# Autodesk Inventor assembly: Rebuild Electrical Board 1
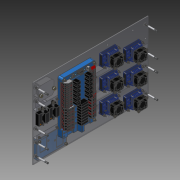
[picture p0: Inventor's stored thumbnail of the model, 180x180]
Saved by Autodesk Inventor 2014 SP1 (Build 180222100, 222)
## iProperties
Created: 2013-01-27
Part Number: Rebuild Electrical Board 1
Document SubType Name: Assembly
Designer: Moses
Mass: 4890.59 g
Surface Area: 13907.1 cm^2
Volume: 1924.91 cm^3
Density: 2.54069 g/cm^3
Author: Moses
## Documents named in this file (25)
- C:\Users\Moses\Documents\Inventor\Sally Rebuild\Rebuild Sally\Rebuild Electrical Board 1.iam
- C:\Users\Moses\Documents\Inventor\Sally Rebuild\Rebuild Sally\CS_PowerBoard_A003206.ipt
- C:\Users\Moses\Documents\Inventor\Sally Rebuild\Rebuild Sally\CS_Converter_CLL25-24S05.ipt
- C:\Users\Moses\Documents\Inventor\Sally Rebuild\Rebuild Sally\93330A493.ipt
- C:\Users\Moses\Documents\Inventor\Sally Rebuild\Rebuild Sally\CS_Relay_SPIKE-RELAY-H.ipt
- C:\Users\Moses\Documents\Inventor\Sally Rebuild\Rebuild Sally\Talon with Fan.iam
- C:\Users\Moses\Documents\Inventor\Sally Rebuild\Rebuild Sally\CS_SideCar_A003333.ipt
- C:\Users\Moses\Documents\Inventor\Sally Rebuild\Rebuild Sally\Rebuild Mounting Board 1.ipt
- C:\Users\Moses\Documents\Inventor\Sally Rebuild\Rebuild Sally\Electrical Board 1 Bracing L Channel.ipt
- C:\Users\Moses\Documents\Inventor\Sally Rebuild\Rebuild Sally\Electrical Board 1 Bracing L Channel Part 2.ipt
- C:\Users\Moses\Documents\Inventor\Sally Rebuild\Rebuild Sally\Pneumatics\Pneumatics_Clippard_AVT-32-32.iam
- C:\Users\Moses\Documents\Inventor\Sally Rebuild\Rebuild Sally\Pneumatics\Pneumatics_SMC_KQ2H07-35S.ipt
- C:\Users\Moses\Documents\Inventor\Sally Rebuild\Rebuild Sally\Standard #10 Washer.ipt
- C:\Users\Moses\Documents\Inventor\Sally Rebuild\Rebuild Sally\10-32 316 Stainless Steel Pan Head Philips Machine Screw\0.500\91735A829.ipt
- C:\Users\Moses\Documents\Inventor\Sally Rebuild\Rebuild Sally\90715A007.ipt
- C:\Users\Moses\Documents\Inventor\Sally Rebuild\Rebuild Sally\6-32 18-8 Stainless Steel Pan Head Philips Machine Screw\0.6250\91772A150.ipt
- C:\Users\Moses\Documents\Inventor\Sally Rebuild\Rebuild Sally\6-32 18-8 Stainless Steel Pan Head Philips Machine Screw\1.0000\91772A153.ipt
- C:\Users\Moses\Documents\Inventor\Sally Rebuild\Rebuild Sally\10-32 316 Stainless Steel Pan Head Philips Machine Screw\0.625\91735A830.ipt
- C:\Users\Moses\Documents\Inventor\Sally Rebuild\Rebuild Sally\6-32 18-8 Stainless Steel Pan Head Philips Machine Screw\1.2500\91772A155.ipt
- C:\Users\Moses\Documents\Inventor\Sally Rebuild\Rebuild Sally\91831A411.ipt
- C:\Users\Moses\Documents\Inventor\Sally Rebuild\Rebuild Sally\Standard #4 Washer.ipt
- C:\Users\Moses\Documents\Inventor\Sally Rebuild\Rebuild Sally\4-40 18-8 Stainless Steel Pan Head Phillips Machine Screw\0.5000\91772A110.ipt
- C:\Users\Moses\Documents\Inventor\Sally Rebuild\Rebuild Sally\4-40 18-8 Stainless Steel Pan Head Phillips Machine Screw\1.1250\91772A118.ipt
- C:\Users\Moses\Documents\Inventor\Sally Rebuild\Rebuild Sally\4-40 18-8 Stainless Steel Pan Head Phillips Machine Screw\18-8 Stainless Steel Machine Screw Hex Nut\91841A005.ipt
- C:\Users\Moses\Documents\Inventor\Sally Rebuild\Rebuild Sally\Standard #6 Washer.ipt
## Components (153 placed, 24 different names)
1. Rebuild Mounting Board 1:1 — Mate:1, Mate:2, Mate:3, Mate:4, Mate:5, Mate:6, Mate:7, Mate:8, Mate:9, Mate:10, Mate:11, Mate:12, Mate:13, Mate:14, Mate:15, Mate:16, Mate:17, Mate:18, Mate:19, Mate:20, Mate:21, Mate:22, Mate:23, Mate:24, Mate:25, Mate:26, Insert:2, Insert:4, Insert:5, Insert:7, Insert:8, Mate:27, Mate:28, Mate:29, Mate:30, Mate:31, Mate:32, Mate:33, Mate:34, Mate:35, Insert:9, Insert:10, Insert:11, Insert:13, Mate:36, Mate:37, Flush:1, Flush:2, Tangent:1, Tangent:2, Flush:5, Flush:6, Mate:38, Mate:39, Insert:18, Insert:19, Insert:20, Insert:21, Insert:22, Insert:23, Insert:24, Insert:25, Insert:26, Angle:3, Angle:4, Insert:90, Insert:91
2. Talon with Fan:1 [sub-assembly] — Mate:1, Mate:6, Mate:7
3. Talon with Fan:2 [sub-assembly] — Mate:2, Mate:8, Mate:9
4. Talon with Fan:3 [sub-assembly] — Mate:3, Mate:10, Mate:11
5. Talon with Fan:4 [sub-assembly] — Mate:4, Mate:12, Mate:13
6. Talon with Fan:5 [sub-assembly] — Mate:14, Mate:15, Mate:16
7. Talon with Fan:6 [sub-assembly] — Mate:5, Mate:17, Mate:18
8. CS_PowerBoard_A003206:1 — Mate:19, Mate:20, Mate:21, Mate:22, Mate:23
9. CS_Converter_CLL25-24S05:1 — Mate:24, Mate:25, Mate:26, Insert:137, Insert:138
10. CS_Relay_SPIKE-RELAY-H:1 — Mate:28, Mate:29, Mate:30
11. CS_Relay_SPIKE-RELAY-H:2 — Mate:27, Mate:31, Mate:32
12. CS_SideCar_A003333:1 — Mate:33, Mate:34, Mate:35
13. Electrical Board 1 Bracing L Channel:1 — Mate:36, Flush:2, Angle:1, Tangent:3, Mate:38, Insert:167
14. Electrical Board 1 Bracing L Channel Part 2:1 — Mate:37, Flush:1, Angle:2, Tangent:4, Mate:39
15. Pneumatics_Clippard_AVT-32-32:1 [sub-assembly] — Tangent:2, Angle:1, Tangent:3, Flush:6, Insert:15, Insert:17, Angle:3
16. Pneumatics_Clippard_AVT-32-32:2 [sub-assembly] — Tangent:1, Angle:2, Tangent:4, Flush:5, Insert:14, Insert:16, Angle:4
17. Pneumatics_SMC_KQ2H07-35S:1 — Insert:14
18. Pneumatics_SMC_KQ2H07-35S:2 — Insert:15
19. Pneumatics_SMC_KQ2H07-35S:3 — Insert:16
20. Pneumatics_SMC_KQ2H07-35S:4 — Insert:17
21. Standard #4 Washer:50 — Insert:133, Insert:167
22. 91841A005:1 — Insert:145
23. 91841A005:2 — Insert:146
24. 91841A005:3 — Insert:147
25. 91841A005:5 — Insert:149
26. 91841A005:4 — Insert:148
27. 91841A005:6 — Insert:150
28. 91841A005:7 — Insert:151
29. 91841A005:8 — Insert:152
30. 91841A005:10 — Insert:153
31. 91841A005:9 — Insert:154
32. 91772A118:2 — Insert:156
33. 91772A118:1 — Insert:155
34. 91772A118:4 — Insert:158
35. 91772A118:3 — Insert:157
36. 91772A118:6 — Insert:160
37. 91772A118:5 — Insert:159
38. 91772A118:7 — Insert:161
39. 91772A118:9 — Insert:163
40. 91772A118:8 — Insert:162
41. 91772A118:10 — Insert:164
42. 91772A118:12 — Insert:166
43. 91772A118:11 — Insert:165
44. 93330A493:2 — Insert:2
45. 93330A493:4 — Insert:4
46. 93330A493:5 — Insert:5
47. 93330A493:7 — Insert:7
48. 93330A493:8 — Insert:8
49. 93330A493:9 — Insert:10
50. 93330A493:11 — Insert:11
51. 93330A493:10 — Insert:9
52. 93330A493:13 — Insert:13
53. 91772A110:1
54. 91772A110:3
55. 91772A110:2
56. 91772A110:4
57. 91772A110:5
58. 91772A110:6
59. 91772A110:7 — Insert:133
60. 91772A110:10
61. 91772A110:8
62. 91772A110:9
63. 91735A830:1 — Insert:137
64. 91735A830:2 — Insert:138
65. 91772A155:1
66. 91772A155:2
67. Standard #4 Washer:49
68. 91772A155:3
69. 91831A411:1 — Insert:143
70. 91831A411:2 — Insert:144
71. 90715A007:5
72. 90715A007:6
73. 90715A007:7
74. 90715A007:8
75. 91772A150:1
76. 91772A150:2
77. 91772A150:3
78. 91772A150:4
79. 90715A007:9
80. 90715A007:11
81. Standard #6 Washer:1
82. Standard #6 Washer:2
83. 91772A153:1
84. 91772A153:2
85. Standard #4 Washer:39 — Insert:151
86. Standard #4 Washer:40 — Insert:152
87. Standard #4 Washer:41 — Insert:154
88. Standard #4 Washer:42 — Insert:153
89. Standard #4 Washer:43 — Insert:145
90. Standard #4 Washer:44 — Insert:150
91. Standard #4 Washer:45 — Insert:146
92. Standard #4 Washer:46 — Insert:149
93. Standard #4 Washer:47 — Insert:148
94. Standard #4 Washer:48 — Insert:147
95. 90715A007:2
96. 90715A007:1
97. 90715A007:4
98. Standard #4 Washer:25 — Insert:157
99. Standard #4 Washer:26 — Insert:158
100. Standard #4 Washer:27 — Insert:155
101. Standard #4 Washer:28 — Insert:156
102. Standard #4 Washer:29 — Insert:161
103. Standard #4 Washer:30 — Insert:162
104. Standard #4 Washer:31 — Insert:160
105. Standard #4 Washer:32 — Insert:159
106. Standard #4 Washer:33 — Insert:164
107. Standard #4 Washer:34 — Insert:163
108. Standard #4 Washer:35 — Insert:166
109. Standard #4 Washer:36 — Insert:165
110. Standard #10 Washer:10 — Insert:91, Insert:143
111. Standard #10 Washer:11 — Insert:90, Insert:144
112. Standard #4 Washer:1
113. Standard #4 Washer:2
114. Standard #4 Washer:3
115. Standard #4 Washer:4
116. Standard #4 Washer:5
117. Standard #4 Washer:6
118. Standard #6 Washer:15
119. Standard #4 Washer:8
120. Standard #6 Washer:12
121. Standard #4 Washer:11
122. Standard #4 Washer:10
123. Standard #6 Washer:8
124. Standard #6 Washer:9
125. Standard #6 Washer:10
126. Standard #6 Washer:11
127. Standard #6 Washer:13
128. Standard #6 Washer:14
129. Standard #6 Washer:7
130. Standard #6 Washer:6
131. Standard #6 Washer:5
132. Standard #6 Washer:4
133. Standard #6 Washer:3
134. Standard #4 Washer:23
135. Standard #4 Washer:24
136. Standard #10 Washer:1 — Insert:18, Insert:27
137. Standard #10 Washer:2 — Insert:19, Insert:28
138. Standard #10 Washer:3 — Insert:20, Insert:29
139. Standard #10 Washer:5 — Insert:22, Insert:31
140. Standard #10 Washer:4 — Insert:21, Insert:30
141. Standard #10 Washer:6 — Insert:23, Insert:32
142. Standard #10 Washer:7 — Insert:24, Insert:33
143. Standard #10 Washer:8 — Insert:25, Insert:34
144. Standard #10 Washer:9 — Insert:26, Insert:35
145. 91735A829:1 — Insert:27
146. 91735A829:2 — Insert:28
147. 91735A829:3 — Insert:29
148. 91735A829:4 — Insert:30
149. 91735A829:5 — Insert:31
150. 91735A829:7 — Insert:33
151. 91735A829:6 — Insert:32
152. 91735A829:8 — Insert:34
153. 91735A829:9 — Insert:35
## Relationships (188: Insert 137, Mate 39, Flush 4, Tangent 4, Angle 4)
- Mate:1: Rebuild Mounting Board 1:1 ↔ Talon with Fan:1
- Mate:2: Rebuild Mounting Board 1:1 ↔ Talon with Fan:2
- Mate:3: Rebuild Mounting Board 1:1 ↔ Talon with Fan:3
- Mate:4: Rebuild Mounting Board 1:1 ↔ Talon with Fan:4
- Mate:5: Rebuild Mounting Board 1:1 ↔ Talon with Fan:6
- Mate:6: Rebuild Mounting Board 1:1 ↔ Talon with Fan:1
- Mate:7: Rebuild Mounting Board 1:1 ↔ Talon with Fan:1
- Mate:8: Rebuild Mounting Board 1:1 ↔ Talon with Fan:2
- Mate:9: Rebuild Mounting Board 1:1 ↔ Talon with Fan:2
- Mate:10: Rebuild Mounting Board 1:1 ↔ Talon with Fan:3
- Mate:11: Rebuild Mounting Board 1:1 ↔ Talon with Fan:3
- Mate:12: Rebuild Mounting Board 1:1 ↔ Talon with Fan:4
- Mate:13: Rebuild Mounting Board 1:1 ↔ Talon with Fan:4
- Mate:14: Rebuild Mounting Board 1:1 ↔ Talon with Fan:5
- Mate:15: Rebuild Mounting Board 1:1 ↔ Talon with Fan:5
- Mate:16: Rebuild Mounting Board 1:1 ↔ Talon with Fan:5
- Mate:17: Rebuild Mounting Board 1:1 ↔ Talon with Fan:6
- Mate:18: Rebuild Mounting Board 1:1 ↔ Talon with Fan:6
- Mate:19: Rebuild Mounting Board 1:1 ↔ CS_PowerBoard_A003206:1
- Mate:20: Rebuild Mounting Board 1:1 ↔ CS_PowerBoard_A003206:1
- Mate:21: Rebuild Mounting Board 1:1 ↔ CS_PowerBoard_A003206:1
- Mate:22: Rebuild Mounting Board 1:1 ↔ CS_PowerBoard_A003206:1
- Mate:23: Rebuild Mounting Board 1:1 ↔ CS_PowerBoard_A003206:1
- Mate:24: Rebuild Mounting Board 1:1 ↔ CS_Converter_CLL25-24S05:1
- Mate:25: Rebuild Mounting Board 1:1 ↔ CS_Converter_CLL25-24S05:1
- Mate:26: Rebuild Mounting Board 1:1 ↔ CS_Converter_CLL25-24S05:1
- Insert:2: Rebuild Mounting Board 1:1 ↔ 93330A493:2
- Insert:4: Rebuild Mounting Board 1:1 ↔ 93330A493:4
- Insert:5: Rebuild Mounting Board 1:1 ↔ 93330A493:5
- Insert:7: Rebuild Mounting Board 1:1 ↔ 93330A493:7
- Insert:8: Rebuild Mounting Board 1:1 ↔ 93330A493:8
- Mate:27: Rebuild Mounting Board 1:1 ↔ CS_Relay_SPIKE-RELAY-H:2
- Mate:28: Rebuild Mounting Board 1:1 ↔ CS_Relay_SPIKE-RELAY-H:1
- Mate:29: Rebuild Mounting Board 1:1 ↔ CS_Relay_SPIKE-RELAY-H:1
- Mate:30: Rebuild Mounting Board 1:1 ↔ CS_Relay_SPIKE-RELAY-H:1
- Mate:31: Rebuild Mounting Board 1:1 ↔ CS_Relay_SPIKE-RELAY-H:2
- Mate:32: Rebuild Mounting Board 1:1 ↔ CS_Relay_SPIKE-RELAY-H:2
- Mate:33: Rebuild Mounting Board 1:1 ↔ CS_SideCar_A003333:1
- Mate:34: Rebuild Mounting Board 1:1 ↔ CS_SideCar_A003333:1
- Mate:35: Rebuild Mounting Board 1:1 ↔ CS_SideCar_A003333:1
- Insert:9: Rebuild Mounting Board 1:1 ↔ 93330A493:10
- Insert:10: Rebuild Mounting Board 1:1 ↔ 93330A493:9
- Insert:11: Rebuild Mounting Board 1:1 ↔ 93330A493:11
- Insert:13: Rebuild Mounting Board 1:1 ↔ 93330A493:13
- Mate:36: Rebuild Mounting Board 1:1 ↔ Electrical Board 1 Bracing L Channel:1
- Mate:37: Rebuild Mounting Board 1:1 ↔ Electrical Board 1 Bracing L Channel Part 2:1
- Flush:1: Rebuild Mounting Board 1:1 ↔ Electrical Board 1 Bracing L Channel Part 2:1
- Flush:2: Rebuild Mounting Board 1:1 ↔ Electrical Board 1 Bracing L Channel:1
- Tangent:1 (3.81 mm): Rebuild Mounting Board 1:1 ↔ Pneumatics_Clippard_AVT-32-32:2
- Tangent:2: Rebuild Mounting Board 1:1 ↔ Pneumatics_Clippard_AVT-32-32:1
- Angle:1 (0 deg): Electrical Board 1 Bracing L Channel:1 ↔ Pneumatics_Clippard_AVT-32-32:1
- Angle:2 (0 deg): Electrical Board 1 Bracing L Channel Part 2:1 ↔ Pneumatics_Clippard_AVT-32-32:2
- Tangent:3: Electrical Board 1 Bracing L Channel:1 ↔ Pneumatics_Clippard_AVT-32-32:1
- Tangent:4: Electrical Board 1 Bracing L Channel Part 2:1 ↔ Pneumatics_Clippard_AVT-32-32:2
- Flush:5 (25.4 mm): Rebuild Mounting Board 1:1 ↔ Pneumatics_Clippard_AVT-32-32:2
- Flush:6 (127 mm): Rebuild Mounting Board 1:1 ↔ Pneumatics_Clippard_AVT-32-32:1
- Insert:14 (1.27 mm): Pneumatics_Clippard_AVT-32-32:2 ↔ Pneumatics_SMC_KQ2H07-35S:1
- Insert:15 (1.27 mm): Pneumatics_Clippard_AVT-32-32:1 ↔ Pneumatics_SMC_KQ2H07-35S:2
- Insert:16 (1.27 mm): Pneumatics_Clippard_AVT-32-32:2 ↔ Pneumatics_SMC_KQ2H07-35S:3
- Insert:17 (1.27 mm): Pneumatics_Clippard_AVT-32-32:1 ↔ Pneumatics_SMC_KQ2H07-35S:4
- Mate:38: Rebuild Mounting Board 1:1 ↔ Electrical Board 1 Bracing L Channel:1
- Mate:39: Rebuild Mounting Board 1:1 ↔ Electrical Board 1 Bracing L Channel Part 2:1
- Insert:18: Rebuild Mounting Board 1:1 ↔ Standard #10 Washer:1
- Insert:19: Rebuild Mounting Board 1:1 ↔ Standard #10 Washer:2
- Insert:20: Rebuild Mounting Board 1:1 ↔ Standard #10 Washer:3
- Insert:21: Rebuild Mounting Board 1:1 ↔ Standard #10 Washer:4
- Insert:22: Rebuild Mounting Board 1:1 ↔ Standard #10 Washer:5
- Insert:23: Rebuild Mounting Board 1:1 ↔ Standard #10 Washer:6
- Insert:24: Rebuild Mounting Board 1:1 ↔ Standard #10 Washer:7
- Insert:25: Rebuild Mounting Board 1:1 ↔ Standard #10 Washer:8
- Insert:26: Rebuild Mounting Board 1:1 ↔ Standard #10 Washer:9
- Insert:27: Standard #10 Washer:1 ↔ 91735A829:1
- Insert:28: Standard #10 Washer:2 ↔ 91735A829:2
- Insert:29: Standard #10 Washer:3 ↔ 91735A829:3
- Insert:30: Standard #10 Washer:4 ↔ 91735A829:4
- Insert:31: Standard #10 Washer:5 ↔ 91735A829:5
- Insert:32: Standard #10 Washer:6 ↔ 91735A829:6
- Insert:33: Standard #10 Washer:7 ↔ 91735A829:7
- Insert:34: Standard #10 Washer:8 ↔ 91735A829:8
- Insert:35: Standard #10 Washer:9 ↔ 91735A829:9
- Angle:3 (0 deg): Rebuild Mounting Board 1:1 ↔ Pneumatics_Clippard_AVT-32-32:1
- Angle:4 (0 deg): Rebuild Mounting Board 1:1 ↔ Pneumatics_Clippard_AVT-32-32:2
- [Insert]: Electrical Board 1 Bracing L Channel:1 ↔ Standard #4 Washer:1
- [Insert]: Electrical Board 1 Bracing L Channel:1 ↔ Standard #4 Washer:2
- [Insert]: Electrical Board 1 Bracing L Channel:1 ↔ Standard #4 Washer:3
- [Insert]: Electrical Board 1 Bracing L Channel Part 2:1 ↔ Standard #4 Washer:4
- [Insert]: Electrical Board 1 Bracing L Channel Part 2:1 ↔ Standard #4 Washer:5
- [Insert]: Electrical Board 1 Bracing L Channel Part 2:1 ↔ Standard #4 Washer:6
- [Insert]: Electrical Board 1 Bracing L Channel:1 ↔ Standard #6 Washer:15
- [Insert]: Electrical Board 1 Bracing L Channel:1 ↔ Standard #4 Washer:8
- [Insert]: Electrical Board 1 Bracing L Channel:1 ↔ Standard #6 Washer:12
- [Insert]: Electrical Board 1 Bracing L Channel Part 2:1 ↔ Standard #4 Washer:10
- [Insert]: Electrical Board 1 Bracing L Channel Part 2:1 ↔ Standard #4 Washer:11
- [Insert]: CS_Relay_SPIKE-RELAY-H:1 ↔ Standard #6 Washer:8
- [Insert]: CS_Relay_SPIKE-RELAY-H:2 ↔ Standard #6 Washer:9
- [Insert]: CS_Relay_SPIKE-RELAY-H:1 ↔ Standard #6 Washer:11
- [Insert]: CS_Relay_SPIKE-RELAY-H:2 ↔ Standard #6 Washer:10
- [Insert]: Rebuild Mounting Board 1:1 ↔ Standard #6 Washer:13
- [Insert]: Rebuild Mounting Board 1:1 ↔ Standard #6 Washer:14
- [Insert]: Rebuild Mounting Board 1:1 ↔ Standard #6 Washer:7
- [Insert]: Rebuild Mounting Board 1:1 ↔ Standard #6 Washer:6
- [Insert]: CS_PowerBoard_A003206:1 ↔ Standard #6 Washer:5
- [Insert]: CS_PowerBoard_A003206:1 ↔ Standard #6 Washer:4
- [Insert]: CS_PowerBoard_A003206:1 ↔ Standard #6 Washer:3
- [Insert]: Rebuild Mounting Board 1:1 ↔ Standard #4 Washer:23
- [Insert]: Rebuild Mounting Board 1:1 ↔ Standard #4 Washer:24
- [Insert]: 90715A007:1 ↔ Standard #6 Washer:3
- [Insert]: 90715A007:2 ↔ Standard #6 Washer:4
- [Insert]: 90715A007:4 ↔ Standard #6 Washer:5
- [Insert]: Rebuild Mounting Board 1:1 ↔ Standard #4 Washer:25
- [Insert]: Electrical Board 1 Bracing L Channel:1 ↔ Standard #4 Washer:26
- [Insert]: Rebuild Mounting Board 1:1 ↔ Standard #4 Washer:27
- [Insert]: Rebuild Mounting Board 1:1 ↔ Standard #4 Washer:28
- [Insert]: Rebuild Mounting Board 1:1 ↔ Standard #4 Washer:29
- [Insert]: Rebuild Mounting Board 1:1 ↔ Standard #4 Washer:30
- [Insert]: Rebuild Mounting Board 1:1 ↔ Standard #4 Washer:31
- [Insert]: Rebuild Mounting Board 1:1 ↔ Standard #4 Washer:32
- [Insert]: Rebuild Mounting Board 1:1 ↔ Standard #4 Washer:33
- [Insert]: Rebuild Mounting Board 1:1 ↔ Standard #4 Washer:34
- [Insert]: Rebuild Mounting Board 1:1 ↔ Standard #4 Washer:35
- [Insert]: Electrical Board 1 Bracing L Channel Part 2:1 ↔ Standard #4 Washer:36
- Insert:90: Rebuild Mounting Board 1:1 ↔ Standard #10 Washer:11
- Insert:91: Rebuild Mounting Board 1:1 ↔ Standard #10 Washer:10
- [Insert]: 90715A007:6 ↔ Standard #6 Washer:12
- [Insert]: 90715A007:5 ↔ Standard #6 Washer:15
- [Insert]: 90715A007:8 ↔ Standard #6 Washer:13
- [Insert]: 90715A007:7 ↔ Standard #6 Washer:14
- [Insert]: 91772A150:2 ↔ Standard #6 Washer:11
- [Insert]: 91772A150:1 ↔ Standard #6 Washer:8
- [Insert]: 91772A150:4 ↔ Standard #6 Washer:9
- [Insert]: 91772A150:3 ↔ Standard #6 Washer:10
- [Insert]: 90715A007:11 ↔ Standard #6 Washer:6
- [Insert]: 90715A007:9 ↔ Standard #6 Washer:7
- [Insert]: CS_SideCar_A003333:1 ↔ Standard #6 Washer:1
- [Insert]: CS_SideCar_A003333:1 ↔ Standard #6 Washer:2
- [Insert]: Standard #6 Washer:1 ↔ 91772A153:1
- [Insert]: Standard #6 Washer:2 ↔ 91772A153:2
- [Insert]: Rebuild Mounting Board 1:1 ↔ Standard #4 Washer:39
- [Insert]: Rebuild Mounting Board 1:1 ↔ Standard #4 Washer:40
- [Insert]: Rebuild Mounting Board 1:1 ↔ Standard #4 Washer:42
- [Insert]: Rebuild Mounting Board 1:1 ↔ Standard #4 Washer:41
- [Insert]: Rebuild Mounting Board 1:1 ↔ Standard #4 Washer:45
- [Insert]: Rebuild Mounting Board 1:1 ↔ Standard #4 Washer:43
- [Insert]: Rebuild Mounting Board 1:1 ↔ Standard #4 Washer:44
- [Insert]: Rebuild Mounting Board 1:1 ↔ Standard #4 Washer:46
- [Insert]: Rebuild Mounting Board 1:1 ↔ Standard #4 Washer:48
- [Insert]: Rebuild Mounting Board 1:1 ↔ Standard #4 Washer:47
- [Insert]: 91772A110:1 ↔ Standard #4 Washer:1
- [Insert]: 91772A110:2 ↔ Standard #4 Washer:2
- [Insert]: 91772A110:3 ↔ Standard #4 Washer:4
- [Insert]: 91772A110:4 ↔ Standard #4 Washer:5
- [Insert]: 91772A110:5 ↔ Standard #4 Washer:3
- [Insert]: 91772A110:6 ↔ Standard #4 Washer:8
- Insert:133: Standard #4 Washer:50 ↔ 91772A110:7
- [Insert]: 91772A110:8 ↔ Standard #4 Washer:6
- [Insert]: 91772A110:9 ↔ Standard #4 Washer:10
- [Insert]: 91772A110:10 ↔ Standard #4 Washer:11
- Insert:137: CS_Converter_CLL25-24S05:1 ↔ 91735A830:1
- Insert:138: CS_Converter_CLL25-24S05:1 ↔ 91735A830:2
- [Insert]: 91772A155:2 ↔ Standard #4 Washer:23
- [Insert]: 91772A155:1 ↔ Standard #4 Washer:24
- [Insert]: Standard #4 Washer:49 ↔ 91772A155:3
- [Insert]: Rebuild Mounting Board 1:1 ↔ Standard #4 Washer:49
- Insert:143: 91831A411:1 ↔ Standard #10 Washer:10
- Insert:144: 91831A411:2 ↔ Standard #10 Washer:11
- Insert:145: 91841A005:1 ↔ Standard #4 Washer:43
- Insert:146: 91841A005:2 ↔ Standard #4 Washer:45
- Insert:147: 91841A005:3 ↔ Standard #4 Washer:48
- Insert:148: 91841A005:4 ↔ Standard #4 Washer:47
- Insert:149: 91841A005:5 ↔ Standard #4 Washer:46
- Insert:150: 91841A005:6 ↔ Standard #4 Washer:44
- Insert:151: 91841A005:7 ↔ Standard #4 Washer:39
- Insert:152: 91841A005:8 ↔ Standard #4 Washer:40
- Insert:153: 91841A005:10 ↔ Standard #4 Washer:42
- Insert:154: 91841A005:9 ↔ Standard #4 Washer:41
- Insert:155: 91772A118:1 ↔ Standard #4 Washer:27
- Insert:156: 91772A118:2 ↔ Standard #4 Washer:28
- Insert:157: 91772A118:3 ↔ Standard #4 Washer:25
- Insert:158: 91772A118:4 ↔ Standard #4 Washer:26
- Insert:159: 91772A118:5 ↔ Standard #4 Washer:32
- Insert:160: 91772A118:6 ↔ Standard #4 Washer:31
- Insert:161: 91772A118:7 ↔ Standard #4 Washer:29
- Insert:162: 91772A118:8 ↔ Standard #4 Washer:30
- Insert:163: 91772A118:9 ↔ Standard #4 Washer:34
- Insert:164: 91772A118:10 ↔ Standard #4 Washer:33
- Insert:165: 91772A118:11 ↔ Standard #4 Washer:36
- Insert:166: 91772A118:12 ↔ Standard #4 Washer:35
- Insert:167: Electrical Board 1 Bracing L Channel:1 ↔ Standard #4 Washer:50
## Named parameters: d195_d194 = 0 mm
